# Autodesk Inventor assembly: Final
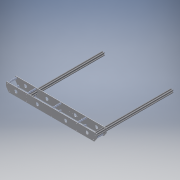
[picture p0: Inventor's stored thumbnail of the model, 180x180]
Saved by Autodesk Inventor 2016 (Build 200138000, 138)
## iProperties
Created: 2017-01-19
Part Number: Final
Document SubType Name: Assembly
Designer: Kyle
Author: Kyle
## Documents named in this file (5)
- C:\Users\Kyle\Documents\FRC1073\FRC1073-CAD\DriveTrain\Final.iam
- C:\Users\Kyle\Documents\FRC1073\FRC1073-CAD\DriveTrain\OutsidePlate.ipt
- C:\Users\Kyle\Documents\FRC1073\FRC1073-CAD\DriveTrain\Individual Parts\Mock 8020 28.25in.ipt
- C:\Users\Kyle\Documents\FRC1073\FRC1073-CAD\DriveTrain\InsidePlate.ipt
- C:\Users\Kyle\Documents\FRC1073\FRC1073-CAD\DriveTrain\Individual Parts\3.625Churro.ipt
## Components (13 placed, 4 different names)
1. OutsidePlate:1 — Mate:1, Mate:2, Flush:1, Flush:2, Mate:3, Flush:3, Flush:4, Mate:4, Mate:5, Mate:6, Mate:7, Mate:8, Mate:9, Mate:10, Mate:11, Mate:12
2. Mock 8020 28.25in:1 — Mate:2, Flush:1, Flush:2
3. Mock 8020 28.25in:2 — Mate:1, Mate:3
4. InsidePlate:1 — Flush:3, Flush:4, Mate:13
5. 3.625Churro:1 — Mate:11
6. 3.625Churro:2 — Mate:10, Mate:13
7. 3.625Churro:3 — Mate:12
8. 3.625Churro:4 — Mate:9
9. 3.625Churro:5 — Mate:7
10. 3.625Churro:6 — Mate:8
11. 3.625Churro:7 — Mate:6
12. 3.625Churro:8 — Mate:4
13. 3.625Churro:9 — Mate:5
## Relationships (17: Mate 13, Flush 4)
- Mate:1: OutsidePlate:1 ↔ Mock 8020 28.25in:2
- Mate:2: OutsidePlate:1 ↔ Mock 8020 28.25in:1
- Flush:1 (6.35 mm): OutsidePlate:1 ↔ Mock 8020 28.25in:1
- Flush:2 (6.35 mm): OutsidePlate:1 ↔ Mock 8020 28.25in:1
- Mate:3: OutsidePlate:1 ↔ Mock 8020 28.25in:2
- Flush:3: OutsidePlate:1 ↔ InsidePlate:1
- Flush:4: OutsidePlate:1 ↔ InsidePlate:1
- Mate:4: OutsidePlate:1 ↔ 3.625Churro:8
- Mate:5: OutsidePlate:1 ↔ 3.625Churro:9
- Mate:6: OutsidePlate:1 ↔ 3.625Churro:7
- Mate:7: OutsidePlate:1 ↔ 3.625Churro:5
- Mate:8: OutsidePlate:1 ↔ 3.625Churro:6
- Mate:9: OutsidePlate:1 ↔ 3.625Churro:4
- Mate:10: OutsidePlate:1 ↔ 3.625Churro:2
- Mate:11: OutsidePlate:1 ↔ 3.625Churro:1
- Mate:12: OutsidePlate:1 ↔ 3.625Churro:3
- Mate:13: InsidePlate:1 ↔ 3.625Churro:2
